# Autodesk Inventor assembly: PitchAssemblyOTS
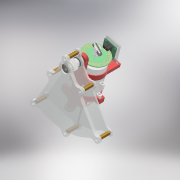
[picture p0: Inventor's stored thumbnail of the model, 180x180]
Saved by Autodesk Inventor 2018.2 (Build 222227000, 227)
## iProperties
Created: 2018-03-26
Part Number: PitchAssemblyOTS
Document SubType Name: Assembly
Designer: mansu
Author: mansu
## Documents named in this file (20)
- C:\Users\Moochster\OneDrive\Documents\2018 UBC\ELEC 391\Controller\cad\release\PitchAssemblyOTS.iam
- C:\Users\Moochster\OneDrive\Documents\2018 UBC\ELEC 391\Controller\cad\release\Rod3_8in.ipt
- C:\Users\Moochster\OneDrive\Documents\2018 UBC\ELEC 391\Controller\cad\release\PitchMotor\pitch_motor_flashlight_attached_model.iam
- C:\Users\Moochster\OneDrive\Documents\2018 UBC\ELEC 391\Controller\cad\release\ShaftArm.ipt
- C:\Users\Moochster\OneDrive\Documents\2018 UBC\ELEC 391\Controller\cad\release\R1038_ZZ_W Bearing.ipt
- C:\Users\Moochster\OneDrive\Documents\2018 UBC\ELEC 391\Controller\cad\release\OmegaRing.ipt
- C:\Users\Moochster\OneDrive\Documents\2018 UBC\ELEC 391\Controller\cad\release\OmegaRingTypeC.ipt
- C:\Users\mansu\Documents\Inventor\Content Center Files\R2018\en-US\AS 1420\AS 1420 - 1973 - M3 x 20.ipt
- C:\Users\mansu\Documents\Inventor\Content Center Files\R2018\en-US\AS 1420\AS 1420 - 1973 - M3 x 14.ipt
- C:\Users\mansu\Documents\Inventor\Content Center Files\R2018\en-US\AS 1474(1)\AS 1474 - M3(1).ipt
- C:\Users\Moochster\OneDrive\Documents\2018 UBC\ELEC 391\Controller\cad\release\RailBase.ipt
- C:\Users\Moochster\OneDrive\Documents\2018 UBC\ELEC 391\Controller\cad\release\EncoderWheelPitch.ipt
- C:\Users\Moochster\OneDrive\Documents\2018 UBC\ELEC 391\Controller\cad\release\EncoderPCBAssembly.iam
- C:\Users\Moochster\OneDrive\Documents\2018 UBC\ELEC 391\Controller\cad\release\EncoderWheelAdapterSmall.ipt
- C:\Users\Moochster\OneDrive\Documents\2018 UBC\ELEC 391\Controller\cad\release\SecondaryEncoderPCBMount.ipt
- C:\Users\Moochster\OneDrive\Documents\2018 UBC\ELEC 391\Controller\cad\release\LaserDiodeAdapter.ipt
- C:\Users\Moochster\OneDrive\Documents\2018 UBC\ELEC 391\Controller\cad\release\VLM-650-03-LPT.ipt
- C:\Users\Moochster\OneDrive\Documents\2018 UBC\ELEC 391\Controller\cad\release\GT2Shaft32T.ipt
- C:\Users\Moochster\OneDrive\Documents\2018 UBC\ELEC 391\Controller\cad\release\Fasteners\StandoffM4x20B.ipt
- C:\Users\Moochster\OneDrive\Documents\2018 UBC\ELEC 391\Controller\cad\release\RailBaseBottom.ipt
## Components (31 placed, 19 different names)
1. Rod3_8in:1 — Mate:9, Mate:10, Flush:2, Mate:29, Mate:43, Mate:44, Mate:46
2. pitch_motor_flashlight_attached_model:1 [sub-assembly] — Mate:14, Mate:18, Mate:19, Mate:20, Insert:1, Insert:2, Insert:3, Mate:22, Mate:24, Mate:26, Mate:28, Angle:1, Mate:30, Mate:31, Mate:34, Mate:40, Flush:4, Angle:4
3. ShaftArm:1 — Mate:10, Mate:11, Flush:1, Mate:15, Mate:16, Flush:2, Angle:1, Mate:35
4. R1038_ZZ_W Bearing:1 — Mate:11, Flush:1, Tangent:3
5. OmegaRingTypeC:1 — Mate:14, Mate:15, Mate:35
6. OmegaRing:2 — Mate:16, Mate:18, Mate:36, Mate:37, Mate:38, Flush:4, Angle:4
7. AS 1420 - Metric M3 x 20:1 — Mate:19, Mate:20, Mate:27
8. AS 1420 - Metric M3 x 20:2 — Insert:1, Mate:21
9. AS 1420 - Metric M3 x 14:1 — Insert:2, Mate:23
10. AS 1420 - Metric M3 x 14:2 — Insert:3, Mate:25
11. AS 1474 - Metric M3:1 — Mate:21, Mate:22
12. AS 1474 - Metric M3:2 — Mate:23, Mate:24
13. AS 1474 - Metric M3:3 — Mate:25, Mate:26
14. AS 1474 - Metric M3:4 — Mate:27, Mate:28
15. RailBase:1 — Mate:29, Flush:5, Tangent:3, Insert:4, Insert:5, Insert:6, Insert:7, Insert:8, Insert:9
16. EncoderWheelPitch:1 — Mate:30, Mate:32, Mate:33, Mate:41, Angle:2
17. EncoderPCBAssembly:1 [sub-assembly] — Tangent:1, Tangent:2, Mate:39, Mate:45
18. EncoderWheelAdapterSmall:1 — Mate:31, Mate:32, Mate:33, Mate:34
19. SecondaryEncoderPCBMount:1 — Mate:36, Mate:37, Mate:38, Tangent:1, Tangent:2, Mate:39, Mate:45
20. LaserDiodeAdapter:1 — Mate:40, Mate:41, Mate:42, Flush:3, Angle:2
21. VLM-650-03-LPT:1 — Mate:42, Flush:3
22. GT2Shaft32T:1 — Mate:43
23. R1038_ZZ_W Bearing:2 — Mate:44, Flush:5
24. StandoffM4x20B:1 — Insert:7
25. StandoffM4x20B:2 — Insert:8
26. StandoffM4x20B:3 — Insert:6
27. StandoffM4x20B:4 — Insert:9
28. StandoffM4x20B:5 — Insert:5, Insert:10
29. StandoffM4x20B:6 — Insert:4
30. R1038_ZZ_W Bearing:3 — Mate:46, Mate:47
31. RailBaseBottom:1 — Mate:47, Insert:10, Angle:3
## Relationships (58: Mate 36, Insert 10, Flush 5, Angle 4, Tangent 3)
- Mate:9: Rod3_8in:1
- Mate:10: Rod3_8in:1 ↔ ShaftArm:1
- Mate:11: ShaftArm:1 ↔ R1038_ZZ_W Bearing:1
- Flush:1 (1 mm): ShaftArm:1 ↔ R1038_ZZ_W Bearing:1
- Mate:14: pitch_motor_flashlight_attached_model:1 ↔ OmegaRingTypeC:1
- Mate:15: ShaftArm:1 ↔ OmegaRingTypeC:1
- Mate:16: ShaftArm:1 ↔ OmegaRing:2
- Flush:2: Rod3_8in:1 ↔ ShaftArm:1
- Mate:18: pitch_motor_flashlight_attached_model:1 ↔ OmegaRing:2
- Mate:19: pitch_motor_flashlight_attached_model:1 ↔ AS 1420 - Metric M3 x 20:1
- Mate:20: pitch_motor_flashlight_attached_model:1 ↔ AS 1420 - Metric M3 x 20:1
- Insert:1: pitch_motor_flashlight_attached_model:1 ↔ AS 1420 - Metric M3 x 20:2
- Insert:2: pitch_motor_flashlight_attached_model:1 ↔ AS 1420 - Metric M3 x 14:1
- Insert:3: pitch_motor_flashlight_attached_model:1 ↔ AS 1420 - Metric M3 x 14:2
- Mate:21: AS 1420 - Metric M3 x 20:2 ↔ AS 1474 - Metric M3:1
- Mate:22: pitch_motor_flashlight_attached_model:1 ↔ AS 1474 - Metric M3:1
- Mate:23: AS 1420 - Metric M3 x 14:1 ↔ AS 1474 - Metric M3:2
- Mate:24: pitch_motor_flashlight_attached_model:1 ↔ AS 1474 - Metric M3:2
- Mate:25: AS 1420 - Metric M3 x 14:2 ↔ AS 1474 - Metric M3:3
- Mate:26: pitch_motor_flashlight_attached_model:1 ↔ AS 1474 - Metric M3:3
- Mate:27: AS 1420 - Metric M3 x 20:1 ↔ AS 1474 - Metric M3:4
- Mate:28: pitch_motor_flashlight_attached_model:1 ↔ AS 1474 - Metric M3:4
- Mate:29: Rod3_8in:1 ↔ RailBase:1
- Angle:1 (0 deg): pitch_motor_flashlight_attached_model:1 ↔ ShaftArm:1
- Mate:30: pitch_motor_flashlight_attached_model:1 ↔ EncoderWheelPitch:1
- Mate:31: pitch_motor_flashlight_attached_model:1 ↔ EncoderWheelAdapterSmall:1
- Mate:32: EncoderWheelPitch:1 ↔ EncoderWheelAdapterSmall:1
- Mate:33 (0.1 mm): EncoderWheelPitch:1 ↔ EncoderWheelAdapterSmall:1
- Mate:34 (0.5 mm): pitch_motor_flashlight_attached_model:1 ↔ EncoderWheelAdapterSmall:1
- Mate:35: ShaftArm:1 ↔ OmegaRingTypeC:1
- Mate:36: OmegaRing:2 ↔ SecondaryEncoderPCBMount:1
- Mate:37: OmegaRing:2 ↔ SecondaryEncoderPCBMount:1
- Mate:38: OmegaRing:2 ↔ SecondaryEncoderPCBMount:1
- Tangent:1: EncoderPCBAssembly:1 ↔ SecondaryEncoderPCBMount:1
- Tangent:2: EncoderPCBAssembly:1 ↔ SecondaryEncoderPCBMount:1
- Mate:39 (3 mm): EncoderPCBAssembly:1 ↔ SecondaryEncoderPCBMount:1
- Mate:40: pitch_motor_flashlight_attached_model:1 ↔ LaserDiodeAdapter:1
- Mate:41 (0.3 mm): EncoderWheelPitch:1 ↔ LaserDiodeAdapter:1
- Mate:42: LaserDiodeAdapter:1 ↔ VLM-650-03-LPT:1
- Flush:3 (-6 mm): LaserDiodeAdapter:1 ↔ VLM-650-03-LPT:1
- Angle:2 (0 deg): EncoderWheelPitch:1 ↔ LaserDiodeAdapter:1
- Flush:4 (-10.5 mm): pitch_motor_flashlight_attached_model:1 ↔ OmegaRing:2
- Mate:43: Rod3_8in:1 ↔ GT2Shaft32T:1
- Mate:44: Rod3_8in:1 ↔ R1038_ZZ_W Bearing:2
- Flush:5 (-0.5 mm): RailBase:1 ↔ R1038_ZZ_W Bearing:2
- Tangent:3 (0.2 mm): R1038_ZZ_W Bearing:1 ↔ RailBase:1
- Mate:45: EncoderPCBAssembly:1 ↔ SecondaryEncoderPCBMount:1
- Insert:4: RailBase:1 ↔ StandoffM4x20B:6
- Insert:5: RailBase:1 ↔ StandoffM4x20B:5
- Insert:6: RailBase:1 ↔ StandoffM4x20B:3
- Insert:7: RailBase:1 ↔ StandoffM4x20B:1
- Insert:8: RailBase:1 ↔ StandoffM4x20B:2
- Insert:9: RailBase:1 ↔ StandoffM4x20B:4
- Mate:46: Rod3_8in:1 ↔ R1038_ZZ_W Bearing:3
- Mate:47: R1038_ZZ_W Bearing:3 ↔ RailBaseBottom:1
- Insert:10: StandoffM4x20B:5 ↔ RailBaseBottom:1
- Angle:3 (0 deg): RailBaseBottom:1
- Angle:4 (0 deg): pitch_motor_flashlight_attached_model:1 ↔ OmegaRing:2
